# Autodesk Inventor assembly: Drive Base Assembly
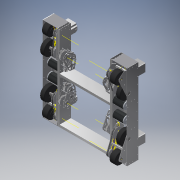
[picture p0: Inventor's stored thumbnail of the model, 180x180]
Saved by Autodesk Inventor 2019.4 (Build 234330000, 330)
## iProperties
Created: 2019-11-02
Part Number: Drive Base Assembly
Document SubType Name: Assembly
Designer: admin
Mass: 32722.2 g
Surface Area: 39593.1 cm^2
Volume: 12105.9 cm^3
Density: 2.70299 g/cm^3
Author: admin
## Documents named in this file (74)
- C:\Users\admin\Desktop\FRC 2020 Engineering\GitHub\7738-CAD-prep\Butterfly Drive Mk2\Butterfly Base\Drive Base Assembly.iam
- C:\Users\admin\Desktop\FRC 2020 Engineering\GitHub\7738-CAD-prep\Butterfly Drive Mk2\Butterfly Base\Main Axle.ipt
- C:\Users\admin\Desktop\FRC 2020 Engineering\GitHub\7738-CAD-prep\Butterfly Drive Mk2\Butterfly Module\Butterfly Drive Module.iam
- C:\Users\admin\Desktop\FRC 2020 Engineering\GitHub\7738-CAD-prep\Butterfly Drive Mk2\Butterfly Base\Side Extrusion.ipt
- C:\Users\admin\Desktop\FRC 2020 Engineering\GitHub\7738-CAD-prep\am-0255 2.5inch CIM Motor.ipt
- C:\Users\admin\Desktop\FRC 2020 Engineering\GitHub\7738-CAD-prep\Butterfly Drive Mk2\Butterfly Base\Mottor Protection Piece.ipt
- C:\Users\admin\Desktop\FRC 2020 Engineering\GitHub\7738-CAD-prep\Butterfly Drive Mk2\Butterfly Base\Drive Base Assembly\Design Accelerator\Spur Gears1.iam
- C:\Users\admin\Desktop\FRC 2020 Engineering\GitHub\7738-CAD-prep\Butterfly Drive Mk2\Butterfly Base\Drive Base Assembly\Design Accelerator\Spur Gears2.iam
- C:\Users\admin\Desktop\FRC 2020 Engineering\GitHub\7738-CAD-prep\Butterfly Drive Mk2\Butterfly Base\Drive Base Assembly\Design Accelerator\Spur Gears3.iam
- C:\Users\admin\Desktop\FRC 2020 Engineering\GitHub\7738-CAD-prep\Butterfly Drive Mk2\Butterfly Base\F6004.ipt
- C:\Users\admin\Desktop\FRC 2020 Engineering\GitHub\7738-CAD-prep\Butterfly Drive Mk2\Butterfly Base\F6802.ipt
- C:\Users\admin\Desktop\FRC 2020 Engineering\GitHub\7738-CAD-prep\Butterfly Drive Mk2\Butterfly Base\F6800Z 10mm ID Flange.ipt
- C:\Users\admin\Desktop\FRC 2020 Engineering\GitHub\7738-CAD-prep\Butterfly Drive Mk2\Butterfly Base\Gearbob Plate.ipt
- C:\Users\admin\Desktop\FRC 2020 Engineering\GitHub\7738-CAD-prep\Butterfly Drive Mk2\Butterfly Base\Gearbob Plate 3mm.ipt
- C:\Users\admin\Desktop\FRC 2020 Engineering\GitHub\7738-CAD-prep\Butterfly Drive Mk2\Butterfly Base\Bumper Plate.ipt
- C:\Users\admin\Desktop\FRC 2020 Engineering\GitHub\7738-CAD-prep\Butterfly Drive Mk2\Butterfly Base\Gearbox Axle 1.ipt
- C:\Users\admin\Desktop\FRC 2020 Engineering\GitHub\7738-CAD-prep\Butterfly Drive Mk2\Butterfly Base\24mm ID Eye bolt.ipt
- C:\Users\admin\Desktop\FRC 2020 Engineering\GitHub\7738-CAD-prep\Butterfly Drive Mk2\Butterfly Base\SDA 63 50 Full.iam
- C:\Users\admin\Desktop\FRC 2020 Engineering\GitHub\7738-CAD-prep\Butterfly drive\Pneumatic Connector.ipt
- C:\Users\admin\Desktop\FRC 2020 Engineering\GitHub\7738-CAD-prep\Butterfly drive\5mm Spacer.ipt
- C:\Users\admin\Desktop\FRC 2020 Engineering\GitHub\7738-CAD-prep\Butterfly Drive Mk2\Butterfly Module\Butterfly Drive Module_MIR.iam
- C:\Users\admin\Desktop\FRC 2020 Engineering\GitHub\7738-CAD-prep\am-0255 2.5inch CIM Motor_MIR.ipt
- C:\Users\admin\Desktop\FRC 2020 Engineering\GitHub\7738-CAD-prep\Butterfly Drive Mk2\Butterfly Base\Drive Base Assembly\Design Accelerator\Spur Gears1_MIR.iam
- C:\Users\admin\Desktop\FRC 2020 Engineering\GitHub\7738-CAD-prep\Butterfly Drive Mk2\Butterfly Base\Drive Base Assembly\Design Accelerator\Spur Gears2_MIR.iam
- C:\Users\admin\Desktop\FRC 2020 Engineering\GitHub\7738-CAD-prep\Butterfly Drive Mk2\Butterfly Base\Drive Base Assembly\Design Accelerator\Spur Gears3_MIR.iam
- C:\Users\admin\Desktop\FRC 2020 Engineering\GitHub\7738-CAD-prep\Butterfly Drive Mk2\Butterfly Base\F6802_MIR.ipt
- C:\Users\admin\Desktop\FRC 2020 Engineering\GitHub\7738-CAD-prep\Butterfly Drive Mk2\Butterfly Base\F6800Z 10mm ID Flange_MIR.ipt
- C:\Users\admin\Desktop\FRC 2020 Engineering\GitHub\7738-CAD-prep\Butterfly Drive Mk2\Butterfly Base\Gearbob Plate_MIR.ipt
- C:\Users\admin\Desktop\FRC 2020 Engineering\GitHub\7738-CAD-prep\Butterfly Drive Mk2\Butterfly Base\Gearbob Plate 3mm_MIR.ipt
- C:\Users\admin\Desktop\FRC 2020 Engineering\GitHub\7738-CAD-prep\Butterfly Drive Mk2\Butterfly Base\F6004_MIR.ipt
- C:\Users\admin\Desktop\FRC 2020 Engineering\GitHub\7738-CAD-prep\Butterfly Drive Mk2\Butterfly Base\Gearbox Axle 1_MIR.ipt
- C:\Users\admin\Desktop\FRC 2020 Engineering\GitHub\7738-CAD-prep\Butterfly Drive Mk2\Butterfly Base\24mm ID Eye bolt_MIR.ipt
- C:\Users\admin\Desktop\FRC 2020 Engineering\GitHub\7738-CAD-prep\Butterfly Drive Mk2\Butterfly Base\SDA 63 50 Full_MIR.iam
- C:\Users\admin\Desktop\FRC 2020 Engineering\GitHub\7738-CAD-prep\Butterfly drive\Pneumatic Connector_MIR1.ipt
- C:\Users\admin\Desktop\FRC 2020 Engineering\GitHub\7738-CAD-prep\Butterfly drive\5mm Spacer_MIR.ipt
- C:\Users\admin\Desktop\FRC 2020 Engineering\GitHub\7738-CAD-prep\Butterfly drive\Vertical Plate Support.ipt
- C:\Users\admin\Desktop\FRC 2020 Engineering\GitHub\7738-CAD-prep\Butterfly drive\Vertical Support Small.ipt
- C:\Users\admin\Desktop\FRC 2020 Engineering\GitHub\7738-CAD-prep\Butterfly Drive Mk2\Butterfly Base\Main Axle_MIR.ipt
- C:\Users\admin\Desktop\FRC 2020 Engineering\GitHub\7738-CAD-prep\Butterfly Drive Mk2\Butterfly Module\Butterfly Drive Module_MIR1.iam
- C:\Users\admin\Desktop\FRC 2020 Engineering\GitHub\7738-CAD-prep\Butterfly Drive Mk2\Butterfly Base\Side Extrusion_MIR.ipt
- C:\Users\admin\Desktop\FRC 2020 Engineering\GitHub\7738-CAD-prep\Butterfly Drive Mk2\Butterfly Base\am-0255 2.5inch CIM Motor_MIR1.ipt
- C:\Users\admin\Desktop\FRC 2020 Engineering\GitHub\7738-CAD-prep\Butterfly Drive Mk2\Butterfly Base\Mottor Protection Piece_MIR1.ipt
- C:\Users\admin\Desktop\FRC 2020 Engineering\GitHub\7738-CAD-prep\Butterfly Drive Mk2\Butterfly Base\Drive Base Assembly\Design Accelerator\Spur Gears1_MIR1.iam
- C:\Users\admin\Desktop\FRC 2020 Engineering\GitHub\7738-CAD-prep\Butterfly Drive Mk2\Butterfly Base\Drive Base Assembly\Design Accelerator\Spur Gears2_MIR1.iam
- C:\Users\admin\Desktop\FRC 2020 Engineering\GitHub\7738-CAD-prep\Butterfly Drive Mk2\Butterfly Base\Drive Base Assembly\Design Accelerator\Spur Gears3_MIR1.iam
- C:\Users\admin\Desktop\FRC 2020 Engineering\GitHub\7738-CAD-prep\Butterfly Drive Mk2\Butterfly Base\F6802_MIR1.ipt
- C:\Users\admin\Desktop\FRC 2020 Engineering\GitHub\7738-CAD-prep\Butterfly Drive Mk2\Butterfly Base\F6800Z 10mm ID Flange_MIR1.ipt
- C:\Users\admin\Desktop\FRC 2020 Engineering\GitHub\7738-CAD-prep\Butterfly Drive Mk2\Butterfly Base\Gearbob Plate_MIR1.ipt
- C:\Users\admin\Desktop\FRC 2020 Engineering\GitHub\7738-CAD-prep\Butterfly Drive Mk2\Butterfly Base\Gearbob Plate 3mm_MIR1.ipt
- C:\Users\admin\Desktop\FRC 2020 Engineering\GitHub\7738-CAD-prep\Butterfly Drive Mk2\Butterfly Base\Bumper Plate_MIR.ipt
- C:\Users\admin\Desktop\FRC 2020 Engineering\GitHub\7738-CAD-prep\Butterfly Drive Mk2\Butterfly Base\F6004_MIR1.ipt
- C:\Users\admin\Desktop\FRC 2020 Engineering\GitHub\7738-CAD-prep\Butterfly Drive Mk2\Butterfly Base\Gearbox Axle 1_MIR1.ipt
- C:\Users\admin\Desktop\FRC 2020 Engineering\GitHub\7738-CAD-prep\Butterfly Drive Mk2\Butterfly Base\24mm ID Eye bolt_MIR1.ipt
- C:\Users\admin\Desktop\FRC 2020 Engineering\GitHub\7738-CAD-prep\Butterfly Drive Mk2\Butterfly Base\SDA 63 50 Full_MIR1.iam
- C:\Users\admin\Desktop\FRC 2020 Engineering\GitHub\7738-CAD-prep\Butterfly drive\Pneumatic Connector_MIR2.ipt
- C:\Users\admin\Desktop\FRC 2020 Engineering\GitHub\7738-CAD-prep\Butterfly drive\5mm Spacer_MIR1.ipt
- C:\Users\admin\Desktop\FRC 2020 Engineering\GitHub\7738-CAD-prep\Butterfly Drive Mk2\Butterfly Module\Butterfly Drive Module_MIR_MIR.iam
- C:\Users\admin\Desktop\FRC 2020 Engineering\GitHub\7738-CAD-prep\Butterfly Drive Mk2\Butterfly Base\am-0255 2.5inch CIM Motor_MIR_MIR.ipt
- C:\Users\admin\Desktop\FRC 2020 Engineering\GitHub\7738-CAD-prep\Butterfly Drive Mk2\Butterfly Base\Drive Base Assembly\Design Accelerator\Spur Gears1_MIR_MIR.iam
- C:\Users\admin\Desktop\FRC 2020 Engineering\GitHub\7738-CAD-prep\Butterfly Drive Mk2\Butterfly Base\Drive Base Assembly\Design Accelerator\Spur Gears2_MIR_MIR.iam
- C:\Users\admin\Desktop\FRC 2020 Engineering\GitHub\7738-CAD-prep\Butterfly Drive Mk2\Butterfly Base\Drive Base Assembly\Design Accelerator\Spur Gears3_MIR_MIR.iam
- C:\Users\admin\Desktop\FRC 2020 Engineering\GitHub\7738-CAD-prep\Butterfly Drive Mk2\Butterfly Base\F6802_MIR_MIR.ipt
- C:\Users\admin\Desktop\FRC 2020 Engineering\GitHub\7738-CAD-prep\Butterfly Drive Mk2\Butterfly Base\F6800Z 10mm ID Flange_MIR_MIR.ipt
- C:\Users\admin\Desktop\FRC 2020 Engineering\GitHub\7738-CAD-prep\Butterfly Drive Mk2\Butterfly Base\Gearbob Plate_MIR_MIR.ipt
- C:\Users\admin\Desktop\FRC 2020 Engineering\GitHub\7738-CAD-prep\Butterfly Drive Mk2\Butterfly Base\Gearbob Plate 3mm_MIR_MIR.ipt
- C:\Users\admin\Desktop\FRC 2020 Engineering\GitHub\7738-CAD-prep\Butterfly Drive Mk2\Butterfly Base\F6004_MIR_MIR.ipt
- C:\Users\admin\Desktop\FRC 2020 Engineering\GitHub\7738-CAD-prep\Butterfly Drive Mk2\Butterfly Base\Gearbox Axle 1_MIR_MIR.ipt
- C:\Users\admin\Desktop\FRC 2020 Engineering\GitHub\7738-CAD-prep\Butterfly Drive Mk2\Butterfly Base\24mm ID Eye bolt_MIR_MIR.ipt
- C:\Users\admin\Desktop\FRC 2020 Engineering\GitHub\7738-CAD-prep\Butterfly Drive Mk2\Butterfly Base\SDA 63 50 Full_MIR_MIR.iam
- C:\Users\admin\Desktop\FRC 2020 Engineering\GitHub\7738-CAD-prep\Butterfly drive\Pneumatic Connector_MIR1_MIR.ipt
- C:\Users\admin\Desktop\FRC 2020 Engineering\GitHub\7738-CAD-prep\Butterfly drive\5mm Spacer_MIR_MIR.ipt
- C:\Users\admin\Desktop\FRC 2020 Engineering\GitHub\7738-CAD-prep\Butterfly drive\Vertical Plate Support_MIR.ipt
- C:\Users\admin\Desktop\FRC 2020 Engineering\GitHub\7738-CAD-prep\Butterfly drive\Vertical Support Small_MIR.ipt
- C:\Users\admin\Desktop\FRC 2020 Engineering\GitHub\7738-CAD-prep\Butterfly drive\Mid.ipt
## Components (120 placed, 71 different names)
1. Main Axle:1 — Mate:28, Mate:29, Mate:49, Mate:52, Mate:63
2. Butterfly Drive Module:1 [sub-assembly] — Mate:63, Mate:64, Angle:3
3. Side Extrusion:1 — Mate:5, Flush:2, Mate:8, Mate:10, Flush:3, Flush:4, Mate:17, Mate:19, Angle:2, Mate:43, Flush:6, Mate:44, Mate:45, Mate:46, Mate:47, Flush:7, Flush:8, Mate:53, Mate:64, Angle:3, Mate:69, Flush:11, Mate:70, Flush:12, Flush:17, Flush:20, Mate:122, Flush:21, Mate:123, Flush:22, Flush:23, Mate:125, Flush:24, Flush:25, Mate:127, Mate:132, Mate:134, Mate:135, Mate:136, Mate:137, Mate:140, Angle:4
4. am-0255 2.5inch CIM Motor:1 — Mate:12, Mate:17, Mate:19, Mate:43, Mate:44
5. Motor Protection Piece:1 — Mate:5, Flush:2, Flush:6, Mate:71, Mate:124, Mate:128, Mate:129, Mate:130, Mate:131
6. Spur Gears:1 [sub-assembly] — Mate:11, Mate:14, Mate:16, Mate:18, Mate:20, Mate:21, Mate:35, Mate:41, Mate:42
7. Spur Gears:2 [sub-assembly] — Mate:8, Mate:11, Mate:18
8. Spur Gears:3 [sub-assembly] — Mate:12, Mate:14, Mate:16
9. F6802:1 — Mate:51, Mate:56
10. F6800Z 10mm ID Flange:1 — Mate:28, Mate:29, Flush:5, Mate:39
11. F6800Z 10mm ID Flange:2 — Mate:35, Flush:5, Mate:38, Mate:57, Flush:9
12. Gearbob Plate:1 — Mate:38, Mate:39, Mate:41, Mate:42, Mate:60, Mate:61, Mate:74, Mate:75, Mate:76, Mate:77, Mate:78, Mate:79, Mate:80, Mate:81, Mate:82, Mate:83
13. Gearbob Plate 3mm:1 — Mate:45, Mate:46, Mate:47, Mate:51, Mate:54, Mate:55, Mate:56, Mate:58, Mate:59
14. Bumper Plate:1 — Flush:7, Flush:8, Mate:50, Mate:66, Flush:20, Mate:122, Mate:126, Mate:138, Flush:26
15. F6802:2 — Mate:49, Mate:50, Mate:66
16. F6004:2 — Mate:52, Mate:53
17. F6800Z 10mm ID Flange:3 — Mate:54, Mate:55
18. Gearbox Axle 1:1 — Mate:57, Flush:9
19. F6800Z 10mm ID Flange:4 — Mate:58, Mate:59
20. F6800Z 10mm ID Flange:5 — Mate:60, Mate:61, Mate:62, Flush:10
21. Gearbox Axle 1:2 — Mate:62, Flush:10
22. 24mm ID Eye bolt:1 — Mate:67, Mate:68
23. SDA 63 50 Full:1 [sub-assembly] — Mate:67, Mate:68, Mate:69, Mate:72, Mate:73
24. Pneumatic Connector:1 — Mate:70, Mate:71, Flush:12, Mate:72, Mate:73
25. 5mm Spacer:1 — Mate:74, Mate:75
26. 5mm Spacer:2 — Mate:76, Mate:77
27. 5mm Spacer:3 — Mate:78, Mate:79
28. 5mm Spacer:4 — Mate:80, Mate:81
29. 5mm Spacer:5 — Mate:82, Mate:83
30. Butterfly Drive Module_MIR:1 [sub-assembly] — Mate:138, Mate:141, Angle:4
31. am-0255 2.5inch CIM Motor_MIR:1 — Mate:88, Mate:134, Mate:135
32. Spur Gears1_MIR:1 [sub-assembly] — Mate:84, Mate:85, Mate:86, Mate:87, Mate:89, Mate:90, Mate:91, Mate:92, Mate:93
33. Spur Gears2_MIR:1 [sub-assembly] — Mate:84, Mate:85
34. Spur Gears3_MIR:1 [sub-assembly] — Mate:86, Mate:87, Mate:88
35. F6802_MIR:1 — Mate:96, Mate:97, Mate:142
36. F6800Z 10mm ID Flange_MIR:1 — Flush:13, Mate:94, Flush:16, Mate:120
37. F6800Z 10mm ID Flange_MIR:2 — Flush:13, Mate:91, Mate:95, Flush:14, Mate:100
38. Gearbob Plate_MIR:1 — Mate:92, Mate:93, Mate:94, Mate:95, Mate:103, Mate:104, Mate:110, Mate:111, Mate:112, Mate:113, Mate:114, Mate:115, Mate:116, Mate:117, Mate:118, Mate:119, Mate:136, Mate:137, Mate:139, Mate:142, Mate:143
39. Gearbob Plate 3mm_MIR:1 — Mate:96, Mate:97, Mate:98, Mate:99, Mate:101, Mate:102, Mate:140
40. F6802_MIR:2
41. F6004_MIR:1
42. F6800Z 10mm ID Flange_MIR:3 — Mate:98, Mate:99
43. Gearbox Axle 1_MIR:1 — Flush:14, Mate:100
44. F6800Z 10mm ID Flange_MIR:4 — Mate:101, Mate:102, Mate:143
45. F6800Z 10mm ID Flange_MIR:5 — Mate:103, Mate:104, Flush:15, Mate:105
46. Gearbox Axle 1_MIR:2 — Flush:15, Mate:105
47. 24mm ID Eye bolt_MIR:1 — Mate:106, Mate:107
48. SDA 63 50 Full_MIR:1 [sub-assembly] — Mate:106, Mate:107, Mate:108, Mate:109, Mate:144
49. Pneumatic Connector_MIR1:1 — Mate:108, Mate:109, Flush:21, Mate:123, Mate:124, Mate:144
50. 5mm Spacer_MIR:1 — Mate:110, Mate:111
51. 5mm Spacer_MIR:2 — Mate:112, Mate:113
52. 5mm Spacer_MIR:3 — Mate:114, Mate:115
53. 5mm Spacer_MIR:4 — Mate:116, Mate:117
54. 5mm Spacer_MIR:5 — Mate:118, Mate:119
55. Main Axle:2 — Flush:16, Mate:120, Mate:139, Mate:141
56. Vertical Plate Support:1 — Flush:22, Flush:23, Mate:125
57. Vertical Plate Support:2 — Flush:24, Mate:126, Flush:25
58. Vertical Support Small:1 — Mate:127, Mate:128, Mate:129
59. Vertical Support Small:2 — Mate:130, Mate:131, Mate:132
60. Main Axle_MIR:1 — Mate:145, Mate:161, Mate:162, Mate:176, Mate:178
61. Butterfly Drive Module_MIR1:1 [sub-assembly] — Mate:145, Mate:146, Angle:6
62. Side Extrusion_MIR:1 — Mate:146, Flush:27, Flush:28, Mate:147, Mate:148, Mate:149, Mate:150, Mate:151, Flush:29, Flush:30, Mate:152, Mate:155, Angle:5, Mate:170, Mate:171, Mate:172, Mate:173, Flush:32, Angle:6, Flush:33, Flush:34, Mate:177, Mate:187, Flush:37, Flush:38, Mate:193, Mate:205, Mate:206, Mate:214, Mate:215, Mate:220, Mate:236, Flush:42, Angle:7, Flush:44, Mate:255, Flush:47, Flush:48, Flush:49, Flush:50, Mate:259, Mate:260, Mate:264, Flush:51, Flush:52, Mate:265, Flush:53
63. am-0255 2.5inch CIM Motor_MIR1:1 — Mate:148, Mate:149, Mate:150, Mate:151, Mate:158
64. Mottor Protection Piece_MIR1:1 — Flush:29, Flush:30, Mate:152, Mate:192, Mate:235, Mate:257, Mate:258, Mate:261, Mate:262
65. Spur Gears1_MIR1:1 [sub-assembly] — Mate:153, Mate:154, Mate:156, Mate:157, Mate:159, Mate:160, Mate:163, Mate:164, Mate:165
66. Spur Gears2_MIR1:1 [sub-assembly] — Mate:153, Mate:154, Mate:155
67. Spur Gears3_MIR1:1 [sub-assembly] — Mate:156, Mate:157, Mate:158
68. F6802_MIR1:1 — Mate:168, Mate:169
69. F6800Z 10mm ID Flange_MIR1:1 — Mate:161, Mate:162, Flush:31, Mate:166
70. F6800Z 10mm ID Flange_MIR1:2 — Flush:31, Mate:163, Mate:167, Flush:35, Mate:181
71. Gearbob Plate_MIR1:1 — Mate:164, Mate:165, Mate:166, Mate:167, Mate:184, Mate:185, Mate:194, Mate:195, Mate:196, Mate:197, Mate:198, Mate:199, Mate:200, Mate:201, Mate:202, Mate:203
72. Gearbob Plate 3mm_MIR1:1 — Mate:168, Mate:169, Mate:170, Mate:171, Mate:172, Mate:179, Mate:180, Mate:182, Mate:183
73. Bumper Plate_MIR:1 — Mate:173, Flush:32, Flush:33, Flush:34, Mate:174, Mate:175, Mate:204, Mate:256, Mate:263
74. F6802_MIR1:2 — Mate:174, Mate:175, Mate:176
75. F6004_MIR1:1 — Mate:177, Mate:178
76. F6800Z 10mm ID Flange_MIR1:3 — Mate:179, Mate:180
77. Gearbox Axle 1_MIR1:1 — Flush:35, Mate:181
78. F6800Z 10mm ID Flange_MIR1:4 — Mate:182, Mate:183
79. F6800Z 10mm ID Flange_MIR1:5 — Mate:184, Mate:185, Flush:36, Mate:186
80. Gearbox Axle 1_MIR1:2 — Flush:36, Mate:186
81. 24mm ID Eye bolt_MIR1:1 — Mate:188, Mate:189
82. SDA 63 50 Full_MIR1:1 [sub-assembly] — Mate:187, Mate:188, Mate:189, Mate:190, Mate:191
83. Pneumatic Connector_MIR2:1 — Mate:190, Mate:191, Flush:38, Mate:192, Mate:193
84. 5mm Spacer_MIR1:1 — Mate:194, Mate:195
85. 5mm Spacer_MIR1:2 — Mate:196, Mate:197
86. 5mm Spacer_MIR1:3 — Mate:198, Mate:199
87. 5mm Spacer_MIR1:4 — Mate:200, Mate:201
88. 5mm Spacer_MIR1:5 — Mate:202, Mate:203
89. Butterfly Drive Module_MIR_MIR:1 [sub-assembly] — Mate:204, Angle:7, Mate:251
90. am-0255 2.5inch CIM Motor_MIR_MIR:1 — Mate:205, Mate:206, Mate:209
91. Spur Gears1_MIR_MIR:1 [sub-assembly] — Mate:207, Mate:208, Mate:210, Mate:211, Mate:212, Mate:218, Mate:219, Mate:249, Mate:250
92. Spur Gears2_MIR_MIR:1 [sub-assembly] — Mate:207, Mate:208
93. Spur Gears3_MIR_MIR:1 [sub-assembly] — Mate:209, Mate:210, Mate:211
94. F6802_MIR_MIR:1 — Mate:213, Mate:221, Mate:222
95. F6800Z 10mm ID Flange_MIR_MIR:1 — Flush:39, Mate:217, Mate:253, Flush:43
96. F6800Z 10mm ID Flange_MIR_MIR:2 — Mate:212, Flush:39, Mate:216, Mate:225, Flush:40
97. Gearbob Plate_MIR_MIR:1 — Mate:213, Mate:214, Mate:215, Mate:216, Mate:217, Mate:218, Mate:219, Mate:226, Mate:229, Mate:230, Mate:239, Mate:240, Mate:241, Mate:242, Mate:243, Mate:244, Mate:245, Mate:246, Mate:247, Mate:248, Mate:252
98. Gearbob Plate 3mm_MIR_MIR:1 — Mate:220, Mate:221, Mate:222, Mate:223, Mate:224, Mate:227, Mate:228
99. F6802_MIR_MIR:2
100. F6004_MIR_MIR:1
101. F6800Z 10mm ID Flange_MIR_MIR:3 — Mate:223, Mate:224
102. Gearbox Axle 1_MIR_MIR:1 — Mate:225, Flush:40
103. F6800Z 10mm ID Flange_MIR_MIR:4 — Mate:226, Mate:227, Mate:228
104. F6800Z 10mm ID Flange_MIR_MIR:5 — Mate:229, Mate:230, Mate:231, Flush:41
105. Gearbox Axle 1_MIR_MIR:2 — Mate:231, Flush:41
106. 24mm ID Eye bolt_MIR_MIR:1 — Mate:232, Mate:233
107. SDA 63 50 Full_MIR_MIR:1 [sub-assembly] — Mate:232, Mate:233, Mate:234, Mate:237, Mate:238
108. Pneumatic Connector_MIR1_MIR:1 — Mate:234, Mate:235, Mate:236, Flush:42, Mate:237, Mate:238
109. 5mm Spacer_MIR_MIR:1 — Mate:239, Mate:240
110. 5mm Spacer_MIR_MIR:2 — Mate:241, Mate:242
111. 5mm Spacer_MIR_MIR:3 — Mate:243, Mate:244
112. 5mm Spacer_MIR_MIR:4 — Mate:245, Mate:246
113. 5mm Spacer_MIR_MIR:5 — Mate:247, Mate:248
114. Main Axle_MIR:2 — Mate:251, Mate:252, Mate:253, Flush:43
115. Vertical Plate Support_MIR:1 — Mate:255, Flush:47, Flush:48
116. Vertical Plate Support_MIR:2 — Flush:49, Mate:256, Flush:50
117. Vertical Support Small_MIR:1 — Mate:257, Mate:258, Mate:259
118. Vertical Support Small_MIR:2 — Mate:260, Mate:261, Mate:262
119. Mid:1 — Mate:264, Flush:51, Flush:52
120. Mid:2 — Mate:265, Flush:53
## Relationships (291: Mate 237, Flush 48, Angle 6)
- Mate:5 (0.5 mm): Side Extrusion:1 ↔ Motor Protection Piece:1
- Flush:2: Side Extrusion:1 ↔ Motor Protection Piece:1
- Mate:8 (7 mm): Side Extrusion:1 ↔ Spur Gears:2
- Mate:10: Side Extrusion:1
- Flush:3: Side Extrusion:1
- Flush:4: Side Extrusion:1
- Mate:11 (5 mm): Spur Gears:1 ↔ Spur Gears:2
- Mate:12: am-0255 2.5inch CIM Motor:1 ↔ Spur Gears:3
- Mate:14 (5 mm): Spur Gears:1 ↔ Spur Gears:3
- Mate:16: Spur Gears:1 ↔ Spur Gears:3
- Mate:17 (0.3 mm): Side Extrusion:1 ↔ am-0255 2.5inch CIM Motor:1
- Mate:18: Spur Gears:1 ↔ Spur Gears:2
- Mate:19: Side Extrusion:1 ↔ am-0255 2.5inch CIM Motor:1
- Mate:20: Spur Gears:1
- Mate:21: Spur Gears:1
- Angle:2 (0 deg): Side Extrusion:1
- Mate:28: Main Axle:1 ↔ F6800Z 10mm ID Flange:1
- Mate:29 (0.3 mm): Main Axle:1 ↔ F6800Z 10mm ID Flange:1
- Mate:35: Spur Gears:1 ↔ F6800Z 10mm ID Flange:2
- Flush:5: F6800Z 10mm ID Flange:1 ↔ F6800Z 10mm ID Flange:2
- Mate:38: F6800Z 10mm ID Flange:2 ↔ Gearbob Plate:1
- Mate:39 (0.3 mm): F6800Z 10mm ID Flange:1 ↔ Gearbob Plate:1
- Mate:41 (4 mm): Spur Gears:1 ↔ Gearbob Plate:1
- Mate:42: Spur Gears:1 ↔ Gearbob Plate:1
- Mate:43: Side Extrusion:1 ↔ am-0255 2.5inch CIM Motor:1
- Flush:6 (270 mm): Side Extrusion:1 ↔ Motor Protection Piece:1
- Mate:44: Side Extrusion:1 ↔ am-0255 2.5inch CIM Motor:1
- Mate:45: Side Extrusion:1 ↔ Gearbob Plate 3mm:1
- Mate:46: Side Extrusion:1 ↔ Gearbob Plate 3mm:1
- Mate:47 (0.2 mm): Side Extrusion:1 ↔ Gearbob Plate 3mm:1
- Flush:7: Side Extrusion:1 ↔ Bumper Plate:1
- Flush:8: Side Extrusion:1 ↔ Bumper Plate:1
- Mate:49: Main Axle:1 ↔ F6802:2
- Mate:50 (0.3 mm): Bumper Plate:1 ↔ F6802:2
- Mate:51 (0.3 mm): F6802:1 ↔ Gearbob Plate 3mm:1
- Mate:52: Main Axle:1 ↔ F6004:2
- Mate:53 (0.3 mm): Side Extrusion:1 ↔ F6004:2
- Mate:54: Gearbob Plate 3mm:1 ↔ F6800Z 10mm ID Flange:3
- Mate:55 (0.3 mm): Gearbob Plate 3mm:1 ↔ F6800Z 10mm ID Flange:3
- Mate:56: F6802:1 ↔ Gearbob Plate 3mm:1
- Mate:57: F6800Z 10mm ID Flange:2 ↔ Gearbox Axle 1:1
- Flush:9: F6800Z 10mm ID Flange:2 ↔ Gearbox Axle 1:1
- Mate:58: Gearbob Plate 3mm:1 ↔ F6800Z 10mm ID Flange:4
- Mate:59 (0.3 mm): Gearbob Plate 3mm:1 ↔ F6800Z 10mm ID Flange:4
- Mate:60 (0.3 mm): Gearbob Plate:1 ↔ F6800Z 10mm ID Flange:5
- Mate:61: Gearbob Plate:1 ↔ F6800Z 10mm ID Flange:5
- Mate:62: F6800Z 10mm ID Flange:5 ↔ Gearbox Axle 1:2
- Flush:10: F6800Z 10mm ID Flange:5 ↔ Gearbox Axle 1:2
- Mate:63: Main Axle:1 ↔ Butterfly Drive Module:1
- Mate:64 (6.5 mm): Butterfly Drive Module:1 ↔ Side Extrusion:1
- Mate:66: Bumper Plate:1 ↔ F6802:2
- Angle:3 (25 deg): Butterfly Drive Module:1 ↔ Side Extrusion:1
- Mate:67: 24mm ID Eye bolt:1 ↔ SDA 63 50 Full:1
- Mate:68 (1 mm): 24mm ID Eye bolt:1 ↔ SDA 63 50 Full:1
- Mate:69 (11 mm): Side Extrusion:1 ↔ SDA 63 50 Full:1
- Flush:11 (-375 mm): Side Extrusion:1
- Mate:70 (0.5 mm): Side Extrusion:1 ↔ Pneumatic Connector:1
- Mate:71 (90 mm): Motor Protection Piece:1 ↔ Pneumatic Connector:1
- Flush:12 (-3 mm): Side Extrusion:1 ↔ Pneumatic Connector:1
- Mate:72: SDA 63 50 Full:1 ↔ Pneumatic Connector:1
- Mate:73: SDA 63 50 Full:1 ↔ Pneumatic Connector:1
- Mate:74: Gearbob Plate:1 ↔ 5mm Spacer:1
- Mate:75 (0.4 mm): Gearbob Plate:1 ↔ 5mm Spacer:1
- Mate:76: Gearbob Plate:1 ↔ 5mm Spacer:2
- Mate:77 (0.4 mm): Gearbob Plate:1 ↔ 5mm Spacer:2
- Mate:78: Gearbob Plate:1 ↔ 5mm Spacer:3
- Mate:79 (0.4 mm): Gearbob Plate:1 ↔ 5mm Spacer:3
- Mate:80: Gearbob Plate:1 ↔ 5mm Spacer:4
- Mate:81 (0.4 mm): Gearbob Plate:1 ↔ 5mm Spacer:4
- Mate:82: Gearbob Plate:1 ↔ 5mm Spacer:5
- Mate:83 (0.4 mm): Gearbob Plate:1 ↔ 5mm Spacer:5
- Mate:84: Spur Gears1_MIR:1 ↔ Spur Gears2_MIR:1
- Mate:85 (5 mm): Spur Gears1_MIR:1 ↔ Spur Gears2_MIR:1
- Mate:86: Spur Gears1_MIR:1 ↔ Spur Gears3_MIR:1
- Mate:87 (5 mm): Spur Gears1_MIR:1 ↔ Spur Gears3_MIR:1
- Mate:88: am-0255 2.5inch CIM Motor_MIR:1 ↔ Spur Gears3_MIR:1
- Mate:89: Spur Gears1_MIR:1
- Mate:90: Spur Gears1_MIR:1
- Flush:13: F6800Z 10mm ID Flange_MIR:1 ↔ F6800Z 10mm ID Flange_MIR:2
- Mate:91: Spur Gears1_MIR:1 ↔ F6800Z 10mm ID Flange_MIR:2
- Mate:92: Spur Gears1_MIR:1 ↔ Gearbob Plate_MIR:1
- Mate:93 (4 mm): Spur Gears1_MIR:1 ↔ Gearbob Plate_MIR:1
- Mate:94 (0.3 mm): F6800Z 10mm ID Flange_MIR:1 ↔ Gearbob Plate_MIR:1
- Mate:95: F6800Z 10mm ID Flange_MIR:2 ↔ Gearbob Plate_MIR:1
- Mate:96: F6802_MIR:1 ↔ Gearbob Plate 3mm_MIR:1
- Mate:97 (0.3 mm): F6802_MIR:1 ↔ Gearbob Plate 3mm_MIR:1
- Mate:98 (0.3 mm): Gearbob Plate 3mm_MIR:1 ↔ F6800Z 10mm ID Flange_MIR:3
- Mate:99: Gearbob Plate 3mm_MIR:1 ↔ F6800Z 10mm ID Flange_MIR:3
- Flush:14: F6800Z 10mm ID Flange_MIR:2 ↔ Gearbox Axle 1_MIR:1
- Mate:100: F6800Z 10mm ID Flange_MIR:2 ↔ Gearbox Axle 1_MIR:1
- Mate:101 (0.3 mm): Gearbob Plate 3mm_MIR:1 ↔ F6800Z 10mm ID Flange_MIR:4
- Mate:102: Gearbob Plate 3mm_MIR:1 ↔ F6800Z 10mm ID Flange_MIR:4
- Mate:103: Gearbob Plate_MIR:1 ↔ F6800Z 10mm ID Flange_MIR:5
- Mate:104 (0.3 mm): Gearbob Plate_MIR:1 ↔ F6800Z 10mm ID Flange_MIR:5
- Flush:15: F6800Z 10mm ID Flange_MIR:5 ↔ Gearbox Axle 1_MIR:2
- Mate:105: F6800Z 10mm ID Flange_MIR:5 ↔ Gearbox Axle 1_MIR:2
- Mate:106 (1 mm): 24mm ID Eye bolt_MIR:1 ↔ SDA 63 50 Full_MIR:1
- Mate:107: 24mm ID Eye bolt_MIR:1 ↔ SDA 63 50 Full_MIR:1
- Mate:108: SDA 63 50 Full_MIR:1 ↔ Pneumatic Connector_MIR1:1
- Mate:109: SDA 63 50 Full_MIR:1 ↔ Pneumatic Connector_MIR1:1
- Mate:110 (0.4 mm): Gearbob Plate_MIR:1 ↔ 5mm Spacer_MIR:1
- Mate:111: Gearbob Plate_MIR:1 ↔ 5mm Spacer_MIR:1
- Mate:112 (0.4 mm): Gearbob Plate_MIR:1 ↔ 5mm Spacer_MIR:2
- Mate:113: Gearbob Plate_MIR:1 ↔ 5mm Spacer_MIR:2
- Mate:114 (0.4 mm): Gearbob Plate_MIR:1 ↔ 5mm Spacer_MIR:3
- Mate:115: Gearbob Plate_MIR:1 ↔ 5mm Spacer_MIR:3
- Mate:116 (0.4 mm): Gearbob Plate_MIR:1 ↔ 5mm Spacer_MIR:4
- Mate:117: Gearbob Plate_MIR:1 ↔ 5mm Spacer_MIR:4
- Mate:118 (0.4 mm): Gearbob Plate_MIR:1 ↔ 5mm Spacer_MIR:5
- Mate:119: Gearbob Plate_MIR:1 ↔ 5mm Spacer_MIR:5
- Flush:16 (0.3 mm): F6800Z 10mm ID Flange_MIR:1 ↔ Main Axle:2
- Mate:120: F6800Z 10mm ID Flange_MIR:1 ↔ Main Axle:2
- Flush:17 (-50 mm): Side Extrusion:1
- Flush:20: Side Extrusion:1 ↔ Bumper Plate:1
- Mate:122 (126 mm): Side Extrusion:1 ↔ Bumper Plate:1
- Flush:21 (-3 mm): Side Extrusion:1 ↔ Pneumatic Connector_MIR1:1
- Mate:123 (0.5 mm): Side Extrusion:1 ↔ Pneumatic Connector_MIR1:1
- Mate:124 (90 mm): Motor Protection Piece:1 ↔ Pneumatic Connector_MIR1:1
- Flush:22: Side Extrusion:1 ↔ Vertical Plate Support:1
- Flush:23: Side Extrusion:1 ↔ Vertical Plate Support:1
- Mate:125 (0.5 mm): Side Extrusion:1 ↔ Vertical Plate Support:1
- Flush:24: Side Extrusion:1 ↔ Vertical Plate Support:2
- Mate:126 (0.5 mm): Bumper Plate:1 ↔ Vertical Plate Support:2
- Flush:25: Side Extrusion:1 ↔ Vertical Plate Support:2
- Mate:127 (0.5 mm): Side Extrusion:1 ↔ Vertical Support Small:1
- Mate:128 (-10 mm): Motor Protection Piece:1 ↔ Vertical Support Small:1
- Mate:129 (0.5 mm): Motor Protection Piece:1 ↔ Vertical Support Small:1
- Mate:130 (-10 mm): Motor Protection Piece:1 ↔ Vertical Support Small:2
- Mate:131 (0.5 mm): Motor Protection Piece:1 ↔ Vertical Support Small:2
- Mate:132 (0.5 mm): Side Extrusion:1 ↔ Vertical Support Small:2
- Mate:134: Side Extrusion:1 ↔ am-0255 2.5inch CIM Motor_MIR:1
- Mate:135: Side Extrusion:1 ↔ am-0255 2.5inch CIM Motor_MIR:1
- Mate:136: Side Extrusion:1 ↔ Gearbob Plate_MIR:1
- Mate:137 (46 mm): Side Extrusion:1 ↔ Gearbob Plate_MIR:1
- Mate:138 (6.5 mm): Bumper Plate:1 ↔ Butterfly Drive Module_MIR:1
- Mate:139: Gearbob Plate_MIR:1 ↔ Main Axle:2
- Mate:140 (0.2 mm): Side Extrusion:1 ↔ Gearbob Plate 3mm_MIR:1
- Mate:141: Butterfly Drive Module_MIR:1 ↔ Main Axle:2
- Mate:142: F6802_MIR:1 ↔ Gearbob Plate_MIR:1
- Mate:143: Gearbob Plate_MIR:1 ↔ F6800Z 10mm ID Flange_MIR:4
- Mate:144 (8 mm): SDA 63 50 Full_MIR:1 ↔ Pneumatic Connector_MIR1:1
- Angle:4 (25 deg): Side Extrusion:1 ↔ Butterfly Drive Module_MIR:1
- Flush:26 (-375 mm): Bumper Plate:1
- Mate:145: Main Axle_MIR:1 ↔ Butterfly Drive Module_MIR1:1
- Mate:146 (6.5 mm): Butterfly Drive Module_MIR1:1 ↔ Side Extrusion_MIR:1
- Flush:27: Side Extrusion_MIR:1
- Flush:28: Side Extrusion_MIR:1
- Mate:147: Side Extrusion_MIR:1
- Mate:148: Side Extrusion_MIR:1 ↔ am-0255 2.5inch CIM Motor_MIR1:1
- Mate:149: Side Extrusion_MIR:1 ↔ am-0255 2.5inch CIM Motor_MIR1:1
- Mate:150: Side Extrusion_MIR:1 ↔ am-0255 2.5inch CIM Motor_MIR1:1
- Mate:151 (0.3 mm): Side Extrusion_MIR:1 ↔ am-0255 2.5inch CIM Motor_MIR1:1
- Flush:29 (270 mm): Side Extrusion_MIR:1 ↔ Mottor Protection Piece_MIR1:1
- Flush:30: Side Extrusion_MIR:1 ↔ Mottor Protection Piece_MIR1:1
- Mate:152 (0.5 mm): Side Extrusion_MIR:1 ↔ Mottor Protection Piece_MIR1:1
- Mate:153: Spur Gears1_MIR1:1 ↔ Spur Gears2_MIR1:1
- Mate:154 (5 mm): Spur Gears1_MIR1:1 ↔ Spur Gears2_MIR1:1
- Mate:155 (7 mm): Side Extrusion_MIR:1 ↔ Spur Gears2_MIR1:1
- Mate:156: Spur Gears1_MIR1:1 ↔ Spur Gears3_MIR1:1
- Mate:157 (5 mm): Spur Gears1_MIR1:1 ↔ Spur Gears3_MIR1:1
- Mate:158: am-0255 2.5inch CIM Motor_MIR1:1 ↔ Spur Gears3_MIR1:1
- Angle:5 (0 deg): Side Extrusion_MIR:1
- Mate:159: Spur Gears1_MIR1:1
- Mate:160: Spur Gears1_MIR1:1
- Mate:161 (0.3 mm): Main Axle_MIR:1 ↔ F6800Z 10mm ID Flange_MIR1:1
- Mate:162: Main Axle_MIR:1 ↔ F6800Z 10mm ID Flange_MIR1:1
- Flush:31: F6800Z 10mm ID Flange_MIR1:1 ↔ F6800Z 10mm ID Flange_MIR1:2
- Mate:163: Spur Gears1_MIR1:1 ↔ F6800Z 10mm ID Flange_MIR1:2
- Mate:164: Spur Gears1_MIR1:1 ↔ Gearbob Plate_MIR1:1
- Mate:165 (4 mm): Spur Gears1_MIR1:1 ↔ Gearbob Plate_MIR1:1
- Mate:166 (0.3 mm): F6800Z 10mm ID Flange_MIR1:1 ↔ Gearbob Plate_MIR1:1
- Mate:167: F6800Z 10mm ID Flange_MIR1:2 ↔ Gearbob Plate_MIR1:1
- Mate:168: F6802_MIR1:1 ↔ Gearbob Plate 3mm_MIR1:1
- Mate:169 (0.3 mm): F6802_MIR1:1 ↔ Gearbob Plate 3mm_MIR1:1
- Mate:170 (0.2 mm): Side Extrusion_MIR:1 ↔ Gearbob Plate 3mm_MIR1:1
- Mate:171: Side Extrusion_MIR:1 ↔ Gearbob Plate 3mm_MIR1:1
- Mate:172: Side Extrusion_MIR:1 ↔ Gearbob Plate 3mm_MIR1:1
- Mate:173 (126 mm): Side Extrusion_MIR:1 ↔ Bumper Plate_MIR:1
- Flush:32: Side Extrusion_MIR:1 ↔ Bumper Plate_MIR:1
- Angle:6 (0 deg): Butterfly Drive Module_MIR1:1 ↔ Side Extrusion_MIR:1
- Flush:33: Side Extrusion_MIR:1 ↔ Bumper Plate_MIR:1
- Flush:34: Side Extrusion_MIR:1 ↔ Bumper Plate_MIR:1
- Mate:174: Bumper Plate_MIR:1 ↔ F6802_MIR1:2
- Mate:175 (0.3 mm): Bumper Plate_MIR:1 ↔ F6802_MIR1:2
- Mate:176: Main Axle_MIR:1 ↔ F6802_MIR1:2
- Mate:177 (0.3 mm): Side Extrusion_MIR:1 ↔ F6004_MIR1:1
- Mate:178: Main Axle_MIR:1 ↔ F6004_MIR1:1
- Mate:179 (0.3 mm): Gearbob Plate 3mm_MIR1:1 ↔ F6800Z 10mm ID Flange_MIR1:3
- Mate:180: Gearbob Plate 3mm_MIR1:1 ↔ F6800Z 10mm ID Flange_MIR1:3
- Flush:35: F6800Z 10mm ID Flange_MIR1:2 ↔ Gearbox Axle 1_MIR1:1
- Mate:181: F6800Z 10mm ID Flange_MIR1:2 ↔ Gearbox Axle 1_MIR1:1
- Mate:182 (0.3 mm): Gearbob Plate 3mm_MIR1:1 ↔ F6800Z 10mm ID Flange_MIR1:4
- Mate:183: Gearbob Plate 3mm_MIR1:1 ↔ F6800Z 10mm ID Flange_MIR1:4
- Mate:184: Gearbob Plate_MIR1:1 ↔ F6800Z 10mm ID Flange_MIR1:5
- Mate:185 (0.3 mm): Gearbob Plate_MIR1:1 ↔ F6800Z 10mm ID Flange_MIR1:5
- Flush:36: F6800Z 10mm ID Flange_MIR1:5 ↔ Gearbox Axle 1_MIR1:2
- Mate:186: F6800Z 10mm ID Flange_MIR1:5 ↔ Gearbox Axle 1_MIR1:2
- Mate:187 (11 mm): Side Extrusion_MIR:1 ↔ SDA 63 50 Full_MIR1:1
- Mate:188 (1 mm): 24mm ID Eye bolt_MIR1:1 ↔ SDA 63 50 Full_MIR1:1
- Mate:189: 24mm ID Eye bolt_MIR1:1 ↔ SDA 63 50 Full_MIR1:1
- Flush:37 (-375 mm): Side Extrusion_MIR:1
- Mate:190: SDA 63 50 Full_MIR1:1 ↔ Pneumatic Connector_MIR2:1
- Mate:191: SDA 63 50 Full_MIR1:1 ↔ Pneumatic Connector_MIR2:1
- Flush:38 (-3 mm): Side Extrusion_MIR:1 ↔ Pneumatic Connector_MIR2:1
- Mate:192 (90 mm): Mottor Protection Piece_MIR1:1 ↔ Pneumatic Connector_MIR2:1
- Mate:193 (0.5 mm): Side Extrusion_MIR:1 ↔ Pneumatic Connector_MIR2:1
- Mate:194 (0.4 mm): Gearbob Plate_MIR1:1 ↔ 5mm Spacer_MIR1:1
- Mate:195: Gearbob Plate_MIR1:1 ↔ 5mm Spacer_MIR1:1
- Mate:196 (0.4 mm): Gearbob Plate_MIR1:1 ↔ 5mm Spacer_MIR1:2
- Mate:197: Gearbob Plate_MIR1:1 ↔ 5mm Spacer_MIR1:2
- Mate:198 (0.4 mm): Gearbob Plate_MIR1:1 ↔ 5mm Spacer_MIR1:3
- Mate:199: Gearbob Plate_MIR1:1 ↔ 5mm Spacer_MIR1:3
- Mate:200 (0.4 mm): Gearbob Plate_MIR1:1 ↔ 5mm Spacer_MIR1:4
- Mate:201: Gearbob Plate_MIR1:1 ↔ 5mm Spacer_MIR1:4
- Mate:202 (0.4 mm): Gearbob Plate_MIR1:1 ↔ 5mm Spacer_MIR1:5
- Mate:203: Gearbob Plate_MIR1:1 ↔ 5mm Spacer_MIR1:5
- Mate:204 (6.5 mm): Bumper Plate_MIR:1 ↔ Butterfly Drive Module_MIR_MIR:1
- Mate:205: Side Extrusion_MIR:1 ↔ am-0255 2.5inch CIM Motor_MIR_MIR:1
- Mate:206: Side Extrusion_MIR:1 ↔ am-0255 2.5inch CIM Motor_MIR_MIR:1
- Mate:207 (5 mm): Spur Gears1_MIR_MIR:1 ↔ Spur Gears2_MIR_MIR:1
- Mate:208: Spur Gears1_MIR_MIR:1 ↔ Spur Gears2_MIR_MIR:1
- Mate:209: am-0255 2.5inch CIM Motor_MIR_MIR:1 ↔ Spur Gears3_MIR_MIR:1
- Mate:210 (5 mm): Spur Gears1_MIR_MIR:1 ↔ Spur Gears3_MIR_MIR:1
- Mate:211: Spur Gears1_MIR_MIR:1 ↔ Spur Gears3_MIR_MIR:1
- Mate:212: Spur Gears1_MIR_MIR:1 ↔ F6800Z 10mm ID Flange_MIR_MIR:2
- Flush:39: F6800Z 10mm ID Flange_MIR_MIR:1 ↔ F6800Z 10mm ID Flange_MIR_MIR:2
- Mate:213: F6802_MIR_MIR:1 ↔ Gearbob Plate_MIR_MIR:1
- Mate:214 (46 mm): Side Extrusion_MIR:1 ↔ Gearbob Plate_MIR_MIR:1
- Mate:215: Side Extrusion_MIR:1 ↔ Gearbob Plate_MIR_MIR:1
- Mate:216: F6800Z 10mm ID Flange_MIR_MIR:2 ↔ Gearbob Plate_MIR_MIR:1
- Mate:217 (0.3 mm): F6800Z 10mm ID Flange_MIR_MIR:1 ↔ Gearbob Plate_MIR_MIR:1
- Mate:218 (4 mm): Spur Gears1_MIR_MIR:1 ↔ Gearbob Plate_MIR_MIR:1
- Mate:219: Spur Gears1_MIR_MIR:1 ↔ Gearbob Plate_MIR_MIR:1
- Mate:220 (0.2 mm): Side Extrusion_MIR:1 ↔ Gearbob Plate 3mm_MIR_MIR:1
- Mate:221 (0.3 mm): F6802_MIR_MIR:1 ↔ Gearbob Plate 3mm_MIR_MIR:1
- Mate:222: F6802_MIR_MIR:1 ↔ Gearbob Plate 3mm_MIR_MIR:1
- Mate:223: Gearbob Plate 3mm_MIR_MIR:1 ↔ F6800Z 10mm ID Flange_MIR_MIR:3
- Mate:224 (0.3 mm): Gearbob Plate 3mm_MIR_MIR:1 ↔ F6800Z 10mm ID Flange_MIR_MIR:3
- Mate:225: F6800Z 10mm ID Flange_MIR_MIR:2 ↔ Gearbox Axle 1_MIR_MIR:1
- Flush:40: F6800Z 10mm ID Flange_MIR_MIR:2 ↔ Gearbox Axle 1_MIR_MIR:1
- Mate:226: Gearbob Plate_MIR_MIR:1 ↔ F6800Z 10mm ID Flange_MIR_MIR:4
- Mate:227: Gearbob Plate 3mm_MIR_MIR:1 ↔ F6800Z 10mm ID Flange_MIR_MIR:4
- Mate:228 (0.3 mm): Gearbob Plate 3mm_MIR_MIR:1 ↔ F6800Z 10mm ID Flange_MIR_MIR:4
- Mate:229 (0.3 mm): Gearbob Plate_MIR_MIR:1 ↔ F6800Z 10mm ID Flange_MIR_MIR:5
- Mate:230: Gearbob Plate_MIR_MIR:1 ↔ F6800Z 10mm ID Flange_MIR_MIR:5
- Mate:231: F6800Z 10mm ID Flange_MIR_MIR:5 ↔ Gearbox Axle 1_MIR_MIR:2
- Flush:41: F6800Z 10mm ID Flange_MIR_MIR:5 ↔ Gearbox Axle 1_MIR_MIR:2
- Mate:232: 24mm ID Eye bolt_MIR_MIR:1 ↔ SDA 63 50 Full_MIR_MIR:1
- Mate:233 (1 mm): 24mm ID Eye bolt_MIR_MIR:1 ↔ SDA 63 50 Full_MIR_MIR:1
- Mate:234 (8 mm): SDA 63 50 Full_MIR_MIR:1 ↔ Pneumatic Connector_MIR1_MIR:1
- Mate:235 (90 mm): Mottor Protection Piece_MIR1:1 ↔ Pneumatic Connector_MIR1_MIR:1
- Mate:236 (0.5 mm): Side Extrusion_MIR:1 ↔ Pneumatic Connector_MIR1_MIR:1
- Flush:42 (-3 mm): Side Extrusion_MIR:1 ↔ Pneumatic Connector_MIR1_MIR:1
- Mate:237: SDA 63 50 Full_MIR_MIR:1 ↔ Pneumatic Connector_MIR1_MIR:1
- Mate:238: SDA 63 50 Full_MIR_MIR:1 ↔ Pneumatic Connector_MIR1_MIR:1
- Mate:239: Gearbob Plate_MIR_MIR:1 ↔ 5mm Spacer_MIR_MIR:1
- Mate:240 (0.4 mm): Gearbob Plate_MIR_MIR:1 ↔ 5mm Spacer_MIR_MIR:1
- Mate:241: Gearbob Plate_MIR_MIR:1 ↔ 5mm Spacer_MIR_MIR:2
- Mate:242 (0.4 mm): Gearbob Plate_MIR_MIR:1 ↔ 5mm Spacer_MIR_MIR:2
- Mate:243: Gearbob Plate_MIR_MIR:1 ↔ 5mm Spacer_MIR_MIR:3
- Mate:244 (0.4 mm): Gearbob Plate_MIR_MIR:1 ↔ 5mm Spacer_MIR_MIR:3
- Mate:245: Gearbob Plate_MIR_MIR:1 ↔ 5mm Spacer_MIR_MIR:4
- Mate:246 (0.4 mm): Gearbob Plate_MIR_MIR:1 ↔ 5mm Spacer_MIR_MIR:4
- Mate:247: Gearbob Plate_MIR_MIR:1 ↔ 5mm Spacer_MIR_MIR:5
- Mate:248 (0.4 mm): Gearbob Plate_MIR_MIR:1 ↔ 5mm Spacer_MIR_MIR:5
- Mate:249: Spur Gears1_MIR_MIR:1
- Mate:250: Spur Gears1_MIR_MIR:1
- Angle:7 (0 deg): Side Extrusion_MIR:1 ↔ Butterfly Drive Module_MIR_MIR:1
- Mate:251: Butterfly Drive Module_MIR_MIR:1 ↔ Main Axle_MIR:2
- Mate:252: Gearbob Plate_MIR_MIR:1 ↔ Main Axle_MIR:2
- Mate:253: F6800Z 10mm ID Flange_MIR_MIR:1 ↔ Main Axle_MIR:2
- Flush:43 (0.3 mm): F6800Z 10mm ID Flange_MIR_MIR:1 ↔ Main Axle_MIR:2
- Flush:44 (-50 mm): Side Extrusion_MIR:1
- Mate:255 (0.5 mm): Side Extrusion_MIR:1 ↔ Vertical Plate Support_MIR:1
- Flush:47: Side Extrusion_MIR:1 ↔ Vertical Plate Support_MIR:1
- Flush:48: Side Extrusion_MIR:1 ↔ Vertical Plate Support_MIR:1
- Flush:49: Side Extrusion_MIR:1 ↔ Vertical Plate Support_MIR:2
- Mate:256 (0.5 mm): Bumper Plate_MIR:1 ↔ Vertical Plate Support_MIR:2
- Flush:50: Side Extrusion_MIR:1 ↔ Vertical Plate Support_MIR:2
- Mate:257 (0.5 mm): Mottor Protection Piece_MIR1:1 ↔ Vertical Support Small_MIR:1
- Mate:258 (-10 mm): Mottor Protection Piece_MIR1:1 ↔ Vertical Support Small_MIR:1
- Mate:259 (0.5 mm): Side Extrusion_MIR:1 ↔ Vertical Support Small_MIR:1
- Mate:260 (0.5 mm): Side Extrusion_MIR:1 ↔ Vertical Support Small_MIR:2
- Mate:261 (0.5 mm): Mottor Protection Piece_MIR1:1 ↔ Vertical Support Small_MIR:2
- Mate:262 (-10 mm): Mottor Protection Piece_MIR1:1 ↔ Vertical Support Small_MIR:2
- Mate:263 (-375 mm): Bumper Plate_MIR:1
- Mate:264: Side Extrusion_MIR:1 ↔ Mid:1
- Flush:51: Side Extrusion_MIR:1 ↔ Mid:1
- Flush:52: Side Extrusion_MIR:1 ↔ Mid:1
- Mate:265: Side Extrusion_MIR:1 ↔ Mid:2
- Flush:53: Side Extrusion_MIR:1 ↔ Mid:2
## Named parameters: Tolerance = 1 mm
